# Autodesk Inventor assembly: Front-Back Component Holds
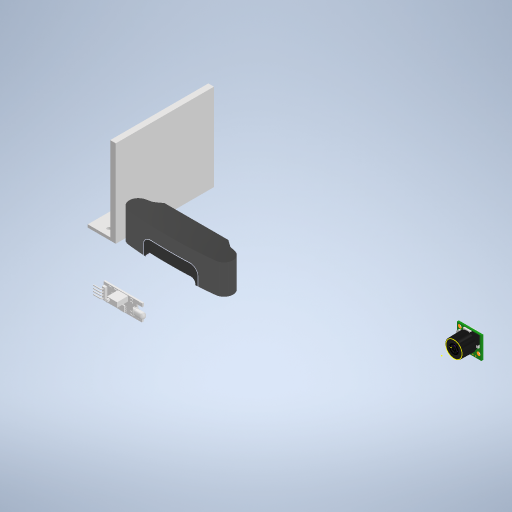
[picture p0: Inventor's stored thumbnail of the model, 512x512]
Saved by Autodesk Inventor 2024 (Build 280153000, 153)
## iProperties
Created: 2024-01-19
Part Number: Front-Back Component Holds
Document SubType Name: Assembly
Designer: Guru
Author: Guru
## Documents named in this file (5)
- D:\Project TRACER\Chassis\Front-Back Component Holds.iam
- D:\Project TRACER\Chassis\Front-Back Hold Plate.ipt
- D:\Project TRACER\IPT Files\TRACERCamera\LogitechC920Montaj.iam
- D:\Project TRACER\IPT Files\KY-026_flame_IR_sensor.ipt
- D:\Project TRACER\IPT Files\XL-MaxSonar-EZ.ipt
## Components (4 placed, 4 different names)
1. Front-Back Hold Plate:1 — Mate:1, Mate:2, Mate:3
2. LogitechC920Montaj:1 [sub-assembly]
3. KY-026_flame_IR_sensor:1
4. XL-MaxSonar-EZ:1
## Relationships (3: Mate 3)
- Mate:1: Front-Back Hold Plate:1
- Mate:2: Front-Back Hold Plate:1
- Mate:3: Front-Back Hold Plate:1
